# Autodesk Inventor assembly: Husky_3D
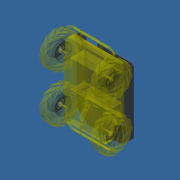
[picture p0: Inventor's stored thumbnail of the model, 180x180]
Saved by Autodesk Inventor 2016 (Build 200138000, 138)
## iProperties
Created: 2021-06-09
Part Number: Husky_3D
Material: Generico
Document SubType Name: Assembly
Designer: Galli Davide
Author: Galli Davide
## Documents named in this file (6)
- C:\Users\galli\OneDrive - Scientific Network South Tyrol\Internship FiRST Lab\Husky_3D_Model\Husky_3D.iam
- C:\Users\galli\OneDrive - Scientific Network South Tyrol\Internship FiRST Lab\Husky_3D_Model\Husky_cover_plate.ipt
- C:\Users\galli\OneDrive - Scientific Network South Tyrol\Internship FiRST Lab\Husky_3D_Model\Husky_top_plate.ipt
- C:\Users\galli\OneDrive\Università\Materie\Mobile Robotics\pozyx_tag_support.ipt
- C:\Users\galli\OneDrive - Scientific Network South Tyrol\Internship FiRST Lab\Husky_3D_Model\Husky_3D_Model_214.ipt
- C:\Users\galli\OneDrive - Scientific Network South Tyrol\Internship FiRST Lab\Husky_3D_Model\Board_cover.ipt
## Components (5 placed, 5 different names)
1. Husky_cover_plate:1 — Perno/foro:1, Perno/foro:2, Perno/foro:3, Angolo:2
2. Husky_top_plate:1 — Perno/foro:1, Perno/foro:2, Coincidente:1, Angolo:1, Allineato:1, Coincidente:2
3. pozyx_tag_support:1 — Perno/foro:3, Angolo:2, Coincidente:3, Coincidente:4, Coincidente:5
4. Husky_3D_Model_214:1 — Coincidente:1, Angolo:1, Allineato:1, Coincidente:2
5. Board_cover:1 — Coincidente:3, Coincidente:4, Coincidente:5
## Relationships (11: Mate 5, Insert 3, Angle 2, Flush 1)
- Perno/foro:1 [Insert]: Husky_cover_plate:1 ↔ Husky_top_plate:1
- Perno/foro:2 [Insert]: Husky_cover_plate:1 ↔ Husky_top_plate:1
- Perno/foro:3 [Insert]: Husky_cover_plate:1 ↔ pozyx_tag_support:1
- Coincidente:1 [Mate]: Husky_top_plate:1 ↔ Husky_3D_Model_214:1
- Angolo:1 [Angle] (0 deg): Husky_top_plate:1 ↔ Husky_3D_Model_214:1
- Allineato:1 [Flush] (100 mm): Husky_top_plate:1 ↔ Husky_3D_Model_214:1
- Coincidente:2 [Mate] (-100 mm): Husky_top_plate:1 ↔ Husky_3D_Model_214:1
- Angolo:2 [Angle] (0 deg): Husky_cover_plate:1 ↔ pozyx_tag_support:1
- Coincidente:3 [Mate]: pozyx_tag_support:1 ↔ Board_cover:1
- Coincidente:4 [Mate] (0.5 mm): pozyx_tag_support:1 ↔ Board_cover:1
- Coincidente:5 [Mate] (0.5 mm): pozyx_tag_support:1 ↔ Board_cover:1
